# Autodesk Inventor assembly: Final_Boss
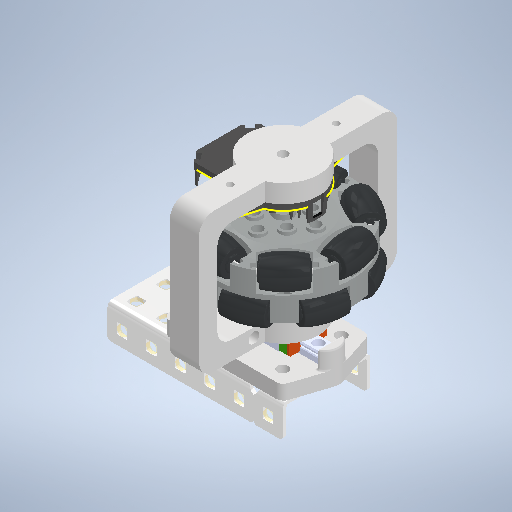
[picture p0: Inventor's stored thumbnail of the model, 512x512]
Saved by Autodesk Inventor 2025.1 (Build 291241020, 241B)
## iProperties
Created: 2024-11-26
Part Number: Final_Boss
Document SubType Name: Assembly
Designer: AtuStem
Author: AtuStem
## Documents named in this file (9)
- C:\Users\AtuStem\Documents\GitHub\ATUM-V5RC-High-Stakes-CAD\Odometers_Collin\Final_Boss.iam
- C:\Users\AtuStem\Documents\GitHub\ATUM-V5RC-High-Stakes-CAD\Odometers_Collin\Linear Rail Files\LinearRail-LWL7B-100mm\LinearRail-LWL7B-100mm\LinearRail-LWL7B-100mm.ipt
- C:\Users\AtuStem\Documents\GitHub\ATUM-V5RC-High-Stakes-CAD\Odometers_Collin\Linear_Odom.ipt
- C:\Users\AtuStem\Documents\GitHub\ATUM-V5RC-High-Stakes-CAD\Odometers_Collin\Linear Rail Files\Carriage-LWL7B\Carriage-LWL7B\Carriage-LWL7B.ipt
- C:\Users\AtuStem\Documents\GitHub\ATUM-V5RC-High-Stakes-CAD\Odometers_Collin\Encoder_Base.ipt
- C:\Users\AtuStem\Documents\GitHub\ATUM-V5RC-High-Stakes-CAD\VEX-CAD-Inventor\Motion\Insert Circle.ipt
- C:\Users\AtuStem\Documents\GitHub\ATUM-V5RC-High-Stakes-CAD\Odometers_Collin\IQ_OMNI.iam
- C:\Users\AtuStem\Documents\GitHub\ATUM-V5RC-High-Stakes-CAD\Odometers_Collin\Linear_Mount.ipt
- C:\Users\AtuStem\Documents\GitHub\ATUM-V5RC-High-Stakes-CAD\VEX-CAD-Inventor\Structure\C Channel\Aluminum 1x3x1\Alu C 1x3x1x6.ipt
## Components (9 placed, 8 different names)
1. LinearRail-LWL7B-100mm:1 — Mate:9, Mate:10, Mate:12, Mate:13
2. Linear_Odom:1 — Mate:1, Flush:4, Mate:16, Flush:5, Mate:18, Mate:19, Mate:20, Mate:21, Mate:22, Mate:23
3. Carriage-LWL7B:1 — Mate:1, Mate:9, Mate:10, Mate:19, Mate:20
4. Linear_Mount:1 — Mate:12, Mate:13, Mate:24, Mate:25
5. Insert Circle:3 — Flush:4, Mate:16, Mate:17
6. Alu C 1x3x1x6:2 — Mate:24, Mate:25
7. IQ_OMNI:2 [sub-assembly] — Mate:17
8. Insert Circle:4 — Flush:5, Mate:18
9. Encoder_Base:1 — Mate:21, Mate:22, Mate:23
## Relationships (17: Mate 15, Flush 2)
- Mate:1: Linear_Odom:1 ↔ Carriage-LWL7B:1
- Mate:9: LinearRail-LWL7B-100mm:1 ↔ Carriage-LWL7B:1
- Mate:10 (0.2032 mm): LinearRail-LWL7B-100mm:1 ↔ Carriage-LWL7B:1
- Mate:12: LinearRail-LWL7B-100mm:1 ↔ Linear_Mount:1
- Mate:13: LinearRail-LWL7B-100mm:1 ↔ Linear_Mount:1
- Flush:4: Linear_Odom:1 ↔ Insert Circle:3
- Mate:16: Linear_Odom:1 ↔ Insert Circle:3
- Mate:17: Insert Circle:3 ↔ IQ_OMNI:2
- Flush:5: Linear_Odom:1 ↔ Insert Circle:4
- Mate:18: Linear_Odom:1 ↔ Insert Circle:4
- Mate:19: Linear_Odom:1 ↔ Carriage-LWL7B:1
- Mate:20: Linear_Odom:1 ↔ Carriage-LWL7B:1
- Mate:21: Linear_Odom:1 ↔ Encoder_Base:1
- Mate:22: Linear_Odom:1 ↔ Encoder_Base:1
- Mate:23: Linear_Odom:1 ↔ Encoder_Base:1
- Mate:24: Linear_Mount:1 ↔ Alu C 1x3x1x6:2
- Mate:25: Linear_Mount:1 ↔ Alu C 1x3x1x6:2
